# Autodesk Inventor assembly: Robot
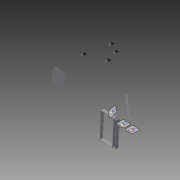
[picture p0: Inventor's stored thumbnail of the model, 180x180]
Saved by Autodesk Inventor 2014 (Build 180170000, 170)
## iProperties
Created: 2014-01-21
Part Number: Robot
Document SubType Name: Assembly
Designer: NilesStanton
Author: NilesStanton
## Documents named in this file (6)
- C:\GitHub\team3566-2014\CAD\Robot.iam
- C:\FIRST-2014-KOP\Drive Base Kit\2014 Sidings.ipt
- C:\FIRST-2014-KOP\Motors\MOT_CIM-Motor_217-2000.iam
- C:\FIRST-2014-KOP\Additions\Flat Board.ipt
- C:\FIRST-2014-KOP\Additions\Front Paneling.ipt
- C:\FIRST-2014-KOP\Additions\3.5 in spacer.ipt
## Components (14 placed, 5 different names)
1. 2014 Sidings:1
2. 2014 Sidings:2 — Mate:2, Flush:2, Mate:4, Flush:4, Angle:1, Flush:5, Angle:3
3. MOT_CIM-Motor_217-2000:1 [sub-assembly]
4. MOT_CIM-Motor_217-2000:2 [sub-assembly]
5. MOT_CIM-Motor_217-2000:3 [sub-assembly]
6. MOT_CIM-Motor_217-2000:4 [sub-assembly]
7. Flat Board:1
8. 2014 Sidings:3
9. Front Paneling:1 — Mate:1, Flush:1, Mate:2, Flush:2, Angle:1
10. Front Paneling:2 — Mate:3, Flush:3, Mate:4, Flush:4, Angle:2, Flush:6
11. 3.5 in spacer:1 — Flush:5, Angle:3, Flush:6, Flush:7, Mate:5, Angle:4
12. 3.5 in spacer:2
13. 2014 Sidings:4 — Flush:7, Mate:5, Angle:4
14. 2014 Sidings:5 — Mate:1, Flush:1, Mate:3, Flush:3, Angle:2
## Relationships (16: Flush 7, Mate 5, Angle 4)
- Mate:1: Front Paneling:1 ↔ 2014 Sidings:5
- Flush:1: Front Paneling:1 ↔ 2014 Sidings:5
- Mate:2: 2014 Sidings:2 ↔ Front Paneling:1
- Flush:2: 2014 Sidings:2 ↔ Front Paneling:1
- Mate:3: Front Paneling:2 ↔ 2014 Sidings:5
- Flush:3: Front Paneling:2 ↔ 2014 Sidings:5
- Mate:4: 2014 Sidings:2 ↔ Front Paneling:2
- Flush:4: 2014 Sidings:2 ↔ Front Paneling:2
- Angle:1 (90 deg): 2014 Sidings:2 ↔ Front Paneling:1
- Angle:2 (90.04 deg): Front Paneling:2 ↔ 2014 Sidings:5
- Flush:5: 2014 Sidings:2 ↔ 3.5 in spacer:1
- Angle:3 (90 deg): 2014 Sidings:2 ↔ 3.5 in spacer:1
- Flush:6: Front Paneling:2 ↔ 3.5 in spacer:1
- Flush:7: 3.5 in spacer:1 ↔ 2014 Sidings:4
- Mate:5: 3.5 in spacer:1 ↔ 2014 Sidings:4
- Angle:4 (270 deg): 3.5 in spacer:1 ↔ 2014 Sidings:4
